# Autodesk Inventor assembly: cortadora
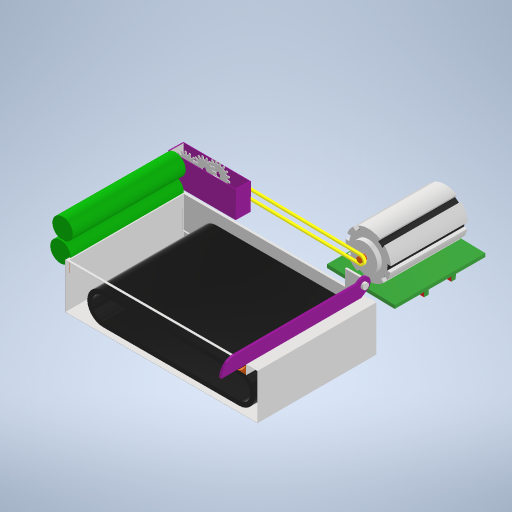
[picture p0: Inventor's stored thumbnail of the model, 512x512]
Saved by Autodesk Inventor 2023 (Build 270158000, 158)
## iProperties
Created: 2022-04-05
Part Number: cortadora
Document SubType Name: Assembly
Designer: isaac
Author: isaac
## Documents named in this file (9)
- C:\Users\isaac\OneDrive\Documentos\Diseño mecánico\cortadora.iam
- C:\Users\isaac\OneDrive\Documentos\Diseño mecánico\banda 1.ipt
- C:\Users\isaac\OneDrive\Documentos\Diseño mecánico\filo.ipt
- C:\Users\isaac\OneDrive\Documentos\Diseño mecánico\cubre.ipt
- C:\Users\isaac\OneDrive\Documentos\Diseño mecánico\rodillo.ipt
- C:\Users\isaac\OneDrive\Documentos\Diseño mecánico\motor.ipt
- C:\Users\isaac\OneDrive\Documentos\Diseño mecánico\faja.ipt
- C:\Users\isaac\OneDrive\Documentos\Diseño mecánico\caja.ipt
- C:\Users\isaac\OneDrive\Documentos\Diseño mecánico\engranaje1.ipt
## Components (11 placed, 8 different names)
1. filo:1 — De rotación:1
2. cubre:1 — De rotación:1, Rígido:1, Coincidencia:1
3. banda 1:1 — Rígido:1
4. rodillo:1 — Coincidencia:1
5. rodillo:2
6. motor:1 — De rotación:2
7. faja:1 — De rotación:2
8. caja:1
9. engranaje1:1
10. engranaje1:2
11. engranaje1:3
## Relationships (4: RevoluteJoint 2, WeldJoint 1, Mate 1)
- De rotación:1 [RevoluteJoint]: filo:1 ↔ cubre:1
- Rígido:1 [WeldJoint]: cubre:1 ↔ banda 1:1
- Coincidencia:1 [Mate] (50 mm): cubre:1 ↔ rodillo:1
- De rotación:2 [RevoluteJoint]: motor:1 ↔ faja:1
